# Autodesk Inventor assembly: Framing_For_First_Floor_Back_Bathroom_Window
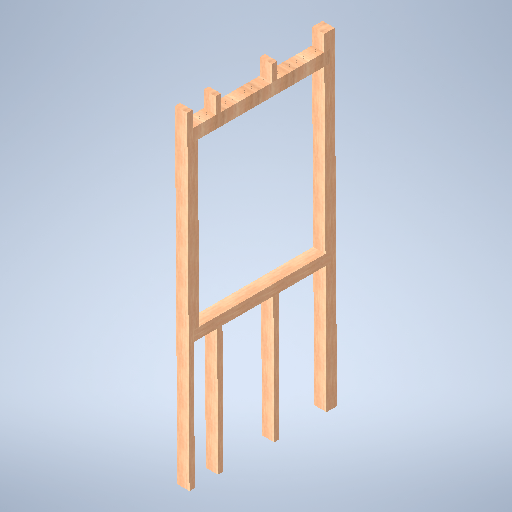
[picture p0: Inventor's stored thumbnail of the model, 512x512]
Saved by Autodesk Inventor 2025.1 (Build 291241020, 241B)
## iProperties
Created: 2024-09-15
Part Number: Framing_For_First_Floor_Back_Bathroom_Window
Document SubType Name: Assembly
Designer: Tom
Author: Tom
## Documents named in this file (7)
- C:\Users\Tom\Documents\Inventor\Mobility\Additional_Building\Framing_For_Bathroom_Window.iam
- C:\Users\Tom\Documents\Inventor\Mobility\Additional_Building\Stud_With_Height_93_Inches.ipt
- C:\Users\Tom\Documents\Inventor\Mobility\Additional_Building\Sill_Plate_With_Length_39_Inches.ipt
- C:\Users\Tom\Documents\Inventor\Mobility\Additional_Building\Stud_With_Height_46_Inches.ipt
- C:\Users\Tom\Documents\Inventor\Mobility\Additional_Building\Header_With_Dimensions_3.5_x_3.5_x_39_Inches.iam
- C:\Users\Tom\Documents\Inventor\Mobility\Additional_Building\Stud_With_Height_4.5625_Inches.ipt
- C:\Users\Tom\Documents\Inventor\Mobility\Additional_Building\Stud_With_Height_35.9375_Inches.ipt
## Components (13 placed, 6 different names)
1. Stud_With_Height_93_Inches:59 — Mate:46, Flush:48, Mate:48, Mate:50, Mate:57, Flush:58, Flush:59, Flush:61, Flush:70, Flush:71, Flush:72
2. Sill_Plate_With_Length_39_Inches:1 — Mate:46, Flush:48, Mate:47, Flush:49, Mate:55, Flush:61, Flush:62, Flush:66, Mate:62, Flush:73
3. Sill_Plate_With_Length_39_Inches:2 — Mate:47, Mate:48, Flush:49, Mate:49, Flush:50, Mate:53, Flush:52, Flush:53, Flush:62, Flush:63, Flush:65
4. Stud_With_Height_46_Inches:1 — Mate:49, Mate:50, Flush:50, Mate:56, Flush:56, Flush:63, Flush:64
5. Stud_With_Height_46_Inches:2 — Mate:53, Flush:52, Flush:53, Flush:65
6. Stud_With_Height_93_Inches:61 — Mate:55, Mate:61, Flush:66, Flush:67, Flush:70, Mate:63
7. Header_With_Dimensions_3.5_x_3.5_x_39_Inches:1 [sub-assembly] — Mate:56, Mate:57, Flush:56, Mate:59, Flush:57, Mate:60, Flush:60, Flush:64, Flush:68, Flush:69
8. Stud_With_Height_4.5625_Inches:3 — Mate:60, Flush:60, Mate:61, Flush:67
9. Stud_With_Height_35.9375_Inches:3 — Mate:62, Flush:73, Mate:63
10. Stud_With_Height_4.5625_Inches:1 — Mate:59, Flush:57, Flush:58, Flush:69
11. Stud_With_Height_4.5625_Inches:2 — Flush:68
12. Stud_With_Height_35.9375_Inches:1 — Flush:59, Flush:71, Flush:72
13. Stud_With_Height_35.9375_Inches:2
## Component patterns: (2 elements, first: Stud_With_Height_4.5625_Inches:1), (2 elements, first: Stud_With_Height_35.9375_Inches:1)
## Relationships (37: Flush 23, Mate 14)
- Mate:46: Stud_With_Height_93_Inches:59 ↔ Sill_Plate_With_Length_39_Inches:1
- Flush:48: Stud_With_Height_93_Inches:59 ↔ Sill_Plate_With_Length_39_Inches:1
- Mate:47: Sill_Plate_With_Length_39_Inches:1 ↔ Sill_Plate_With_Length_39_Inches:2
- Mate:48: Stud_With_Height_93_Inches:59 ↔ Sill_Plate_With_Length_39_Inches:2
- Flush:49: Sill_Plate_With_Length_39_Inches:1 ↔ Sill_Plate_With_Length_39_Inches:2
- Mate:49: Sill_Plate_With_Length_39_Inches:2 ↔ Stud_With_Height_46_Inches:1
- Mate:50: Stud_With_Height_93_Inches:59 ↔ Stud_With_Height_46_Inches:1
- Flush:50: Sill_Plate_With_Length_39_Inches:2 ↔ Stud_With_Height_46_Inches:1
- Mate:53: Sill_Plate_With_Length_39_Inches:2 ↔ Stud_With_Height_46_Inches:2
- Flush:52: Sill_Plate_With_Length_39_Inches:2 ↔ Stud_With_Height_46_Inches:2
- Flush:53: Sill_Plate_With_Length_39_Inches:2 ↔ Stud_With_Height_46_Inches:2
- Mate:55: Sill_Plate_With_Length_39_Inches:1 ↔ Stud_With_Height_93_Inches:61
- Mate:56: Stud_With_Height_46_Inches:1 ↔ Header_With_Dimensions_3.5_x_3.5_x_39_Inches:1
- Mate:57: Stud_With_Height_93_Inches:59 ↔ Header_With_Dimensions_3.5_x_3.5_x_39_Inches:1
- Flush:56: Stud_With_Height_46_Inches:1 ↔ Header_With_Dimensions_3.5_x_3.5_x_39_Inches:1
- Mate:59: Header_With_Dimensions_3.5_x_3.5_x_39_Inches:1 ↔ Stud_With_Height_4.5625_Inches:1
- Flush:57: Header_With_Dimensions_3.5_x_3.5_x_39_Inches:1 ↔ Stud_With_Height_4.5625_Inches:1
- Flush:58 (206.375 mm): Stud_With_Height_93_Inches:59 ↔ Stud_With_Height_4.5625_Inches:1
- Flush:59 (206.375 mm): Stud_With_Height_93_Inches:59 ↔ Stud_With_Height_35.9375_Inches:1
- Mate:60: Header_With_Dimensions_3.5_x_3.5_x_39_Inches:1 ↔ Stud_With_Height_4.5625_Inches:3
- Flush:60: Header_With_Dimensions_3.5_x_3.5_x_39_Inches:1 ↔ Stud_With_Height_4.5625_Inches:3
- Mate:61: Stud_With_Height_93_Inches:61 ↔ Stud_With_Height_4.5625_Inches:3
- Flush:61: Stud_With_Height_93_Inches:59 ↔ Sill_Plate_With_Length_39_Inches:1
- Flush:62: Sill_Plate_With_Length_39_Inches:1 ↔ Sill_Plate_With_Length_39_Inches:2
- Flush:63: Sill_Plate_With_Length_39_Inches:2 ↔ Stud_With_Height_46_Inches:1
- Flush:64: Stud_With_Height_46_Inches:1 ↔ Header_With_Dimensions_3.5_x_3.5_x_39_Inches:1
- Flush:65: Sill_Plate_With_Length_39_Inches:2 ↔ Stud_With_Height_46_Inches:2
- Flush:66: Sill_Plate_With_Length_39_Inches:1 ↔ Stud_With_Height_93_Inches:61
- Flush:67: Stud_With_Height_93_Inches:61 ↔ Stud_With_Height_4.5625_Inches:3
- Flush:68: Header_With_Dimensions_3.5_x_3.5_x_39_Inches:1 ↔ Stud_With_Height_4.5625_Inches:2
- Flush:69: Header_With_Dimensions_3.5_x_3.5_x_39_Inches:1 ↔ Stud_With_Height_4.5625_Inches:1
- Flush:70: Stud_With_Height_93_Inches:59 ↔ Stud_With_Height_93_Inches:61
- Flush:71: Stud_With_Height_93_Inches:59 ↔ Stud_With_Height_35.9375_Inches:1
- Flush:72: Stud_With_Height_93_Inches:59 ↔ Stud_With_Height_35.9375_Inches:1
- Mate:62: Sill_Plate_With_Length_39_Inches:1 ↔ Stud_With_Height_35.9375_Inches:3
- Flush:73: Sill_Plate_With_Length_39_Inches:1 ↔ Stud_With_Height_35.9375_Inches:3
- Mate:63: Stud_With_Height_93_Inches:61 ↔ Stud_With_Height_35.9375_Inches:3
